# Autodesk Inventor assembly: Table
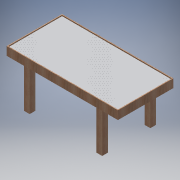
[picture p0: Inventor's stored thumbnail of the model, 180x180]
Saved by Autodesk Inventor 2019.3 (Build 233278000, 278)
## iProperties
Created: 2020-08-13
Part Number: Table
Material: Generisch
Document SubType Name: Assembly
Designer: Nicolas Frick
Author: Nicolas Frick
## Documents named in this file (4)
- C:\Users\Nicolas Frick\Sync\OneDrive\airhockeybot\mechanical_design\inventor\Table.iam
- C:\Users\Nicolas Frick\Sync\OneDrive\airhockeybot\mechanical_design\inventor\Frame.ipt
- C:\Users\Nicolas Frick\Sync\OneDrive\airhockeybot\mechanical_design\inventor\Plate.ipt
- C:\Users\Nicolas Frick\Sync\OneDrive\airhockeybot\mechanical_design\inventor\Leg.ipt
## Components (6 placed, 3 different names)
1. Frame:1 — Passend:1, Passend:2, Fluchtend:1, Passend:7, Passend:8, Passend:9, Passend:10, Passend:11, Passend:12, Passend:13, Passend:14
2. Plate:1 — Passend:1, Passend:2, Fluchtend:1, Passend:3, Passend:4, Passend:5, Passend:6
3. Leg:1 — Passend:4, Passend:7, Passend:12
4. Leg:2 — Passend:5, Passend:8, Passend:11
5. Leg:3 — Passend:6, Passend:10, Passend:14
6. Leg:4 — Passend:3, Passend:9, Passend:13
## Relationships (15: Mate 14, Flush 1)
- Passend:1 [Mate]: Frame:1 ↔ Plate:1
- Passend:2 [Mate]: Frame:1 ↔ Plate:1
- Fluchtend:1 [Flush] (16.5 mm): Frame:1 ↔ Plate:1
- Passend:3 [Mate]: Plate:1 ↔ Leg:4
- Passend:4 [Mate]: Plate:1 ↔ Leg:1
- Passend:5 [Mate]: Plate:1 ↔ Leg:2
- Passend:6 [Mate]: Plate:1 ↔ Leg:3
- Passend:7 [Mate]: Frame:1 ↔ Leg:1
- Passend:8 [Mate]: Frame:1 ↔ Leg:2
- Passend:9 [Mate]: Frame:1 ↔ Leg:4
- Passend:10 [Mate]: Frame:1 ↔ Leg:3
- Passend:11 [Mate] (259 mm): Frame:1 ↔ Leg:2
- Passend:12 [Mate] (259 mm): Frame:1 ↔ Leg:1
- Passend:13 [Mate] (259 mm): Frame:1 ↔ Leg:4
- Passend:14 [Mate] (259 mm): Frame:1 ↔ Leg:3
